# Autodesk Inventor assembly: LIA0006-ARDUINO SHELF
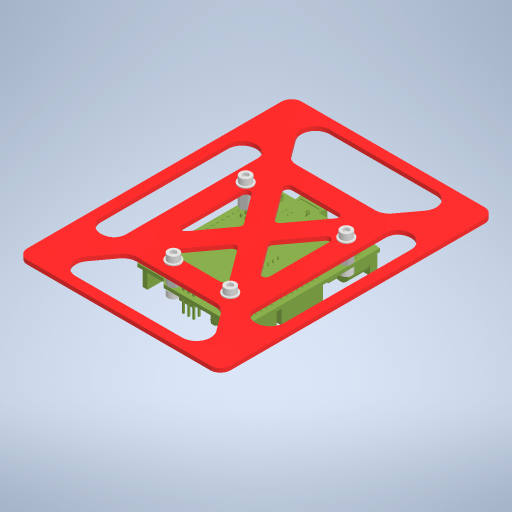
[picture p0: Inventor's stored thumbnail of the model, 512x512]
Saved by Autodesk Inventor 2023 (Build 270158000, 158)
## iProperties
Created: 2023-05-05
Part Number: LIA0006-ARDUINO SHELF
Document SubType Name: Assembly
Designer: Louis
Author: Louis
## Documents named in this file (7)
- D:\Louis\Documents\Inventor\Interferometry\LIA0006-ARDUINO SHELF.iam
- D:\Louis\Documents\Inventor\Interferometry\LI0014-ARDUINO SHELF.ipt
- D:\Louis\Documents\Inventor\Interferometry\ACCU HHTPS-M3-5-8-S-Z.ipt
- D:\Louis\Documents\Inventor\Interferometry\M3 X 6.ipt
- D:\Louis\Documents\Inventor\Interferometry\M3 WASHER.ipt
- D:\Louis\Documents\Inventor\Interferometry\arduino uno_Simplify_1.ipt
- D:\Louis\Documents\Inventor\Interferometry\LI0016-ARDUINO DIE.ipt
## Components (19 placed, 6 different names)
1. LI0014-ARDUINO SHELF:1 — Mate:1, Mate:2, Mate:3, Insert:1, Insert:2, Insert:3, Insert:4, Insert:12, Insert:13, Insert:14, Insert:15
2. M3 X 6:1 — Insert:9
3. M3 X 6:2 — Insert:10
4. M3 X 6:3 — Insert:11
5. M3 X 6:4 — Mate:4
6. M3 X 6:5 — Mate:5
7. M3 X 6:6 — Insert:8
8. M3 WASHER:1 — Insert:15, Mate:7
9. M3 WASHER:2 — Insert:14, Mate:6
10. M3 WASHER:3 — Insert:13, Mate:5
11. M3 WASHER:4 — Insert:12, Mate:4
12. ACCU HHTPS-M3-5-8-S-Z:1 — Insert:1, Insert:6
13. ACCU HHTPS-M3-5-8-S-Z:2 — Insert:3, Insert:5
14. ACCU HHTPS-M3-5-8-S-Z:3 — Insert:4
15. ACCU HHTPS-M3-5-8-S-Z:4 — Insert:2, Insert:7
16. arduino uno_Simplify_1:1 — Insert:5, Insert:6, Insert:7, Insert:8, Insert:9, Insert:10, Insert:11, Mate:8, Flush:1, Flush:2
17. M3 X 6:7 — Mate:6
18. M3 X 6:8 — Mate:7
19. LI0016-ARDUINO DIE:1 — Mate:8, Flush:1, Flush:2
## Relationships (25: Insert 15, Mate 8, Flush 2)
- Mate:1: LI0014-ARDUINO SHELF:1
- Mate:2: LI0014-ARDUINO SHELF:1
- Mate:3: LI0014-ARDUINO SHELF:1
- Insert:1: LI0014-ARDUINO SHELF:1 ↔ ACCU HHTPS-M3-5-8-S-Z:1
- Insert:2: LI0014-ARDUINO SHELF:1 ↔ ACCU HHTPS-M3-5-8-S-Z:4
- Insert:3: LI0014-ARDUINO SHELF:1 ↔ ACCU HHTPS-M3-5-8-S-Z:2
- Insert:4: LI0014-ARDUINO SHELF:1 ↔ ACCU HHTPS-M3-5-8-S-Z:3
- Insert:5: ACCU HHTPS-M3-5-8-S-Z:2 ↔ arduino uno_Simplify_1:1
- Insert:6: ACCU HHTPS-M3-5-8-S-Z:1 ↔ arduino uno_Simplify_1:1
- Insert:7: ACCU HHTPS-M3-5-8-S-Z:4 ↔ arduino uno_Simplify_1:1
- Insert:8: M3 X 6:6 ↔ arduino uno_Simplify_1:1
- Insert:9: M3 X 6:1 ↔ arduino uno_Simplify_1:1
- Insert:10: M3 X 6:2 ↔ arduino uno_Simplify_1:1
- Insert:11: M3 X 6:3 ↔ arduino uno_Simplify_1:1
- Insert:12: LI0014-ARDUINO SHELF:1 ↔ M3 WASHER:4
- Insert:13: LI0014-ARDUINO SHELF:1 ↔ M3 WASHER:3
- Insert:14: LI0014-ARDUINO SHELF:1 ↔ M3 WASHER:2
- Insert:15: LI0014-ARDUINO SHELF:1 ↔ M3 WASHER:1
- Mate:4: M3 X 6:4 ↔ M3 WASHER:4
- Mate:5: M3 X 6:5 ↔ M3 WASHER:3
- Mate:6: M3 WASHER:2 ↔ M3 X 6:7
- Mate:7: M3 WASHER:1 ↔ M3 X 6:8
- Mate:8: arduino uno_Simplify_1:1 ↔ LI0016-ARDUINO DIE:1
- Flush:1 (40 mm): arduino uno_Simplify_1:1 ↔ LI0016-ARDUINO DIE:1
- Flush:2 (10 mm): arduino uno_Simplify_1:1 ↔ LI0016-ARDUINO DIE:1
